# Autodesk Inventor assembly: 自動販賣機3.1
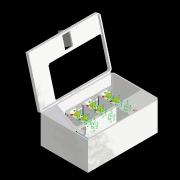
[picture p0: Inventor's stored thumbnail of the model, 180x180]
Saved by Autodesk Inventor 2020 (Build 240168000, 168)
## iProperties
Created: 2021-04-08
Part Number: 自動販賣機3.1
Document SubType Name: Assembly
Designer: 88690
Author: 88690
## Documents named in this file (33)
- C:\Users\88690\Desktop\自動販賣機\自動販賣機3.1.iam
- C:\Users\88690\Desktop\自動販賣機\上滑軌.ipt
- C:\Users\88690\Desktop\自動販賣機\上滑軌輪.ipt
- C:\Users\88690\Desktop\自動販賣機\下滑軌.ipt
- C:\Users\88690\Desktop\自動販賣機\下滑軌輪.ipt
- C:\Users\88690\Desktop\自動販賣機\本體.ipt
- C:\Users\88690\Desktop\自動販賣機\置物架.ipt
- C:\Users\88690\Desktop\自動販賣機\滾筒.ipt
- C:\Users\88690\Desktop\自動販賣機\蓋.ipt
- C:\Users\88690\Desktop\自動販賣機\鎖點支架.ipt
- C:\Users\88690\Desktop\自動販賣機\下支架右.ipt
- C:\Users\88690\Desktop\自動販賣機\上滑軌右.ipt
- C:\Users\88690\Desktop\自動販賣機\蝸桿支架.ipt
- C:\Users\88690\Desktop\自動販賣機\蝸桿滑塊.ipt
- C:\Users\88690\Desktop\自動販賣機\短蝸桿.ipt
- C:\Users\88690\Desktop\自動販賣機\長蝸桿.ipt
- C:\Users\88690\Desktop\自動販賣機\位移平台.ipt
- C:\Users\88690\Desktop\自動販賣機\取物窗.ipt
- C:\Users\88690\Desktop\自動販賣機\螺旋鉤子.ipt
- C:\Users\88690\Desktop\自動販賣機\螺旋鉤子底座.ipt
- C:\Users\88690\Desktop\自動販賣機\名牌1.ipt
- C:\Users\88690\Desktop\自動販賣機\名牌2.ipt
- C:\Users\88690\Desktop\自動販賣機\名牌3.ipt
- C:\Users\88690\Desktop\自動販賣機\名牌4.ipt
- C:\Users\88690\Desktop\自動販賣機\名牌5.ipt
- C:\Users\88690\Desktop\自動販賣機\名牌6.ipt
- C:\Users\88690\Desktop\自動販賣機\名牌7.ipt
- C:\Users\88690\Desktop\自動販賣機\名牌8.ipt
- C:\Users\88690\Desktop\自動販賣機\名牌9.ipt
- C:\Users\88690\Desktop\自動販賣機\模擬商品.ipt
- C:\Users\88690\Desktop\自動販賣機\模擬錢幣.ipt
- C:\Users\88690\Desktop\自動販賣機\路徑2.0.ipt
- C:\Users\88690\Desktop\自動販賣機\商品支架.ipt
## Components (117 placed, 32 different names)
1. 上滑軌:1 — 貼合:41, 貼合:42, 貼合:45, 相切:7, 貼合:183
2. 上滑軌輪:1 — 貼合:41, 貼合:42, 相切:1
3. 下滑軌:1 — 貼合:11, 貼合:12, 貼合:13, 貼合:15, 相切:1, 角度:40
4. 下滑軌輪:1 — 貼合:11, 貼合:12, 相切:7
5. 本體:1 — 齊平:1, 齊平:2, 齊平:3, 貼合:1, 貼合:2, 貼合:3, 貼合:4, 貼合:6, 貼合:7, 貼合:8, 貼合:9, 貼合:75, 貼合:76, 貼合:77, 貼合:78, 貼合:79, 貼合:80, 貼合:81, 貼合:82, 貼合:83, 貼合:84, 貼合:85, 貼合:86, 貼合:88, 貼合:89, 貼合:101, 齊平:23, 角度:1, 旋轉:1, 貼合:167, 角度:34, 貼合:169, 貼合:171, 貼合:172, 貼合:174, 齊平:50, 齊平:51, 貼合:177, 貼合:179, 齊平:53
6. 置物架:1 — 貼合:45, 貼合:50, 貼合:51, 齊平:12, 齊平:13, 貼合:111, 貼合:114, 貼合:131, 貼合:132, 貼合:139, 貼合:143, 貼合:144, 貼合:145, 貼合:146, 旋轉:2, 旋轉:3, 旋轉:10, 齊平:53, 齊平:54, 角度:40, 貼合:183, 角度:41, 貼合:187, 貼合:218, 貼合:219, 貼合:220, 貼合:221, 貼合:222, 貼合:223, 貼合:224
7. 滾筒:1 — 貼合:75, 貼合:76, 齊平:14, 齊平:15, 齊平:16, 齊平:17, 齊平:18, 齊平:19, 齊平:20, 齊平:21, 齊平:22, 角度:12, 旋轉:1, 旋轉:1, 貼合:178, 貼合:180
8. 蓋:1 — 貼合:101, 齊平:23, 角度:1, 角度:2, 貼合:108, 貼合:164, 角度:34, 角度:35
9. 鎖點支架:1 — 貼合:1, 貼合:2, 貼合:3, 齊平:4, 齊平:5, 齊平:6, 齊平:7, 貼合:5, 貼合:15, 貼合:22, 貼合:25
10. 鎖點支架:2 — 齊平:5, 齊平:7, 貼合:5, 貼合:13, 貼合:20, 貼合:23, 貼合:51, 貼合:72, 貼合:165, 貼合:166
11. 鎖點支架:3 — 齊平:4, 齊平:6, 貼合:4
12. 鎖點支架:4 — 齊平:8, 齊平:10, 貼合:9
13. 鎖點支架:5 — 貼合:6, 貼合:7, 貼合:8, 齊平:8, 齊平:9, 齊平:10, 齊平:11, 貼合:10, 貼合:30, 貼合:37, 貼合:40
14. 鎖點支架:6 — 齊平:9, 齊平:11, 貼合:10, 貼合:28, 貼合:35, 貼合:38
15. 下滑軌:2 — 貼合:20, 貼合:22, 相切:4
16. 下滑軌輪:2 — 相切:8
17. 下滑軌:3 — 貼合:23, 貼合:25, 相切:6
18. 下滑軌輪:3 — 相切:9
19. 下支架右:1 — 貼合:26, 貼合:27, 貼合:28, 貼合:30, 相切:2, 貼合:74, 角度:41
20. 下滑軌輪:4 — 貼合:26, 貼合:27, 相切:10
21. 下支架右:2 — 貼合:35, 貼合:37, 相切:3, 角度:42
22. 下滑軌輪:5 — 相切:11
23. 下支架右:3 — 貼合:38, 貼合:40, 相切:5, 角度:43
24. 下滑軌輪:6 — 相切:12
25. 上滑軌右:1 — 貼合:46, 貼合:50, 相切:10, 貼合:186, 貼合:187
26. 上滑軌輪:2 — 貼合:46, 相切:2, 貼合:74, 貼合:186
27. 上滑軌:2 — 相切:8, 貼合:184
28. 上滑軌輪:3 — 相切:4
29. 置物架:2 — 齊平:12, 貼合:72, 貼合:133, 貼合:134, 貼合:135, 貼合:140, 貼合:147, 貼合:150, 貼合:151, 貼合:152, 旋轉:4, 旋轉:5, 旋轉:9, 貼合:165, 齊平:54, 齊平:55, 貼合:184, 角度:42, 貼合:188, 貼合:225, 貼合:226, 貼合:227, 貼合:228, 貼合:229, 貼合:230
30. 上滑軌右:2 — 相切:11, 貼合:188
31. 上滑軌輪:4 — 相切:3
32. 上滑軌:3 — 相切:9, 貼合:185
33. 上滑軌輪:5 — 相切:6
34. 置物架:3 — 齊平:13, 貼合:136, 貼合:137, 貼合:138, 貼合:141, 貼合:148, 貼合:149, 貼合:153, 貼合:154, 旋轉:6, 旋轉:7, 旋轉:8, 貼合:166, 齊平:55, 貼合:185, 角度:43, 貼合:189, 貼合:231, 貼合:232, 貼合:233, 貼合:234, 貼合:235, 貼合:236
35. 上滑軌右:3 — 相切:12, 貼合:189
36. 上滑軌輪:6 — 相切:5
37. 滾筒:2 — 齊平:14, 貼合:77, 旋轉:1, 旋轉:2, 角度:13
38. 滾筒:3 — 齊平:15, 貼合:78, 旋轉:2, 角度:14, 旋轉:3
39. 滾筒:4 — 齊平:16, 貼合:79, 角度:15, 旋轉:3, 旋轉:4
40. 滾筒:5 — 齊平:17, 貼合:80, 角度:16, 旋轉:4, 旋轉:5
41. 滾筒:6 — 齊平:18, 貼合:81, 角度:18, 旋轉:5, 旋轉:6
42. 滾筒:7 — 齊平:19, 貼合:82, 角度:19, 旋轉:6, 旋轉:7
43. 滾筒:8 — 齊平:20, 貼合:83, 角度:22, 旋轉:7, 旋轉:8
44. 滾筒:9 — 齊平:21, 貼合:84, 角度:20, 旋轉:8, 旋轉:9
45. 滾筒:10 — 齊平:22, 貼合:85, 角度:21, 旋轉:9
46. 蝸桿支架:1 — 貼合:86, 貼合:88, 貼合:89, 貼合:90, 貼合:91, 貼合:92, 貼合:93
47. 蝸桿滑塊:1 — 貼合:90, 貼合:91, 貼合:94, 貼合:95, 貼合:97, 貼合:98, 貼合:99
48. 短蝸桿:1 — 貼合:94, 貼合:95, 旋轉/轉換:1
49. 長蝸桿:1 — 貼合:92, 貼合:93, 角度:23, 旋轉/轉換:1
50. 位移平台:1 — 貼合:97, 貼合:98, 貼合:99, 貼合:167, 貼合:182
51. 取物窗:1 — 角度:2, 貼合:108, 貼合:164, 角度:35
52. 螺旋鉤子:1 — 貼合:111, 貼合:112, 貼合:113, 角度:3, 貼合:155, 貼合:191, 貼合:199, 貼合:209
53. 螺旋鉤子底座:1 — 貼合:112, 貼合:113, 貼合:114, 貼合:155, 旋轉:2
54. 螺旋鉤子:2 — 貼合:131, 齊平:44, 貼合:190, 貼合:198, 貼合:208
55. 螺旋鉤子底座:2 — 齊平:25, 貼合:139, 齊平:44, 旋轉:3
56. 螺旋鉤子:3 — 貼合:132, 齊平:47, 貼合:197, 貼合:200, 貼合:210
57. 螺旋鉤子底座:3 — 齊平:25, 齊平:47, 旋轉:10
58. 螺旋鉤子:4 — 貼合:133, 貼合:157, 貼合:192, 貼合:201, 貼合:211, 齊平:96
59. 螺旋鉤子底座:4 — 齊平:26, 齊平:27, 貼合:140, 貼合:157, 旋轉:4
60. 螺旋鉤子:5 — 貼合:134, 貼合:158, 貼合:168, 貼合:170, 角度:37, 齊平:49, 貼合:202, 貼合:207, 貼合:212, 貼合:217, 齊平:96
61. 螺旋鉤子底座:5 — 齊平:26, 貼合:158, 旋轉:5
62. 螺旋鉤子:6 — 貼合:135, 齊平:46, 貼合:193, 貼合:203, 貼合:213
63. 螺旋鉤子底座:6 — 齊平:27, 齊平:46, 旋轉:9
64. 螺旋鉤子:7 — 貼合:136, 貼合:160, 貼合:194, 貼合:204, 貼合:214
65. 螺旋鉤子底座:7 — 齊平:28, 齊平:29, 貼合:141, 貼合:160, 旋轉:6
66. 螺旋鉤子:8 — 貼合:137, 貼合:161, 貼合:195, 貼合:205, 貼合:215
67. 螺旋鉤子底座:8 — 齊平:28, 貼合:161, 旋轉:7
68. 螺旋鉤子:9 — 貼合:138, 齊平:45, 貼合:196, 貼合:206, 貼合:216
69. 螺旋鉤子底座:9 — 齊平:29, 齊平:45, 旋轉:8
70. 名牌1:1 — 貼合:143, 貼合:144, 角度:24, 齊平:30, 角度:25, 角度:29
71. 名牌2:1 — 貼合:145, 齊平:30, 齊平:31, 角度:25, 角度:26
72. 名牌3:1 — 貼合:146, 齊平:31, 角度:26
73. 名牌4:1 — 齊平:32, 齊平:33, 貼合:147, 貼合:150, 角度:27, 角度:28, 角度:29
74. 名牌5:1 — 齊平:32, 貼合:151, 角度:27
75. 名牌6:1 — 齊平:33, 貼合:152, 角度:32
76. 名牌7:1 — 齊平:34, 貼合:148, 貼合:149, 角度:28
77. 名牌8:1 — 齊平:34, 齊平:35, 貼合:153, 角度:30
78. 名牌9:1 — 齊平:35, 貼合:154, 角度:33
79. 模擬商品:1 — 貼合:168, 角度:36, 貼合:170, 角度:38, 貼合:176, 貼合:177, 貼合:178, 貼合:181, 貼合:182, 齊平:63
80. 模擬錢幣:1 — 貼合:169, 貼合:171, 貼合:172
81. 路徑2.0:1 — 貼合:174, 貼合:176, 角度:39, 齊平:50, 齊平:51
82. 路徑2.0:2 — 貼合:179, 貼合:180, 齊平:52, 貼合:181
83. 模擬商品:2 — 貼合:190, 齊平:56, 齊平:57, 齊平:58, 齊平:59, 齊平:60, 齊平:61, 齊平:62, 齊平:63
84. 模擬商品:3 — 貼合:191, 齊平:56
85. 模擬商品:4 — 貼合:192, 齊平:58
86. 模擬商品:5 — 貼合:193, 齊平:59
87. 模擬商品:6 — 貼合:194, 齊平:62
88. 模擬商品:7 — 貼合:197, 齊平:57
89. 模擬商品:8 — 貼合:195, 齊平:61
90. 模擬商品:9 — 貼合:196, 齊平:60
91. 模擬商品:10 — 齊平:83, 貼合:202, 貼合:207
92. 模擬商品:11 — 齊平:80, 齊平:81, 齊平:82, 齊平:83, 齊平:84, 齊平:85, 齊平:86, 齊平:87, 貼合:198
93. 模擬商品:12 — 齊平:80, 貼合:199
94. 模擬商品:13 — 齊平:82, 貼合:201
95. 模擬商品:14 — 齊平:84, 貼合:203
96. 模擬商品:15 — 齊平:85, 貼合:204
97. 模擬商品:16 — 齊平:81, 貼合:200
98. 模擬商品:17 — 齊平:86, 貼合:205
99. 模擬商品:18 — 齊平:87, 貼合:206
100. 模擬商品:19 — 齊平:91, 貼合:212, 貼合:217
101. 模擬商品:20 — 齊平:88, 齊平:90, 齊平:91, 齊平:92, 齊平:93, 齊平:94, 齊平:95, 貼合:208
102. 模擬商品:21 — 齊平:88, 齊平:89, 貼合:209
103. 模擬商品:22 — 齊平:90, 貼合:211
104. 模擬商品:23 — 齊平:92, 貼合:213
105. 模擬商品:24 — 齊平:93, 貼合:214
106. 模擬商品:25 — 齊平:89, 貼合:210
107. 模擬商品:26 — 齊平:94, 貼合:215
108. 模擬商品:27 — 齊平:95, 貼合:216
109. 商品支架:1 — 貼合:218, 貼合:219, 貼合:220, 齊平:103
110. 商品支架:2 — 齊平:97, 貼合:221, 貼合:222, 齊平:103, 齊平:104
111. 商品支架:3 — 齊平:97, 齊平:98, 貼合:225, 貼合:226
112. 商品支架:4 — 齊平:98, 齊平:99, 貼合:235, 貼合:236
113. 商品支架:5 — 齊平:99, 齊平:100, 貼合:227, 貼合:228
114. 商品支架:6 — 齊平:100, 齊平:101, 貼合:229, 貼合:230
115. 商品支架:7 — 齊平:101, 齊平:102, 貼合:231, 貼合:232
116. 商品支架:8 — 貼合:223, 貼合:224, 齊平:104
117. 商品支架:9 — 齊平:102, 貼合:233, 貼合:234
## Relationships (357: Mate 198, Flush 94, Angle 33, Tangent 12, RevoluteJoint 10, RelateRotation 9, RelateRotateTranslate 1)
- 齊平:1 [Flush]: 本體:1
- 齊平:2 [Flush]: 本體:1
- 齊平:3 [Flush]: 本體:1
- 貼合:1 [Mate] (180 mm): 本體:1 ↔ 鎖點支架:1
- 貼合:2 [Mate]: 本體:1 ↔ 鎖點支架:1
- 貼合:3 [Mate]: 本體:1 ↔ 鎖點支架:1
- 齊平:4 [Flush]: 鎖點支架:1 ↔ 鎖點支架:3
- 齊平:5 [Flush]: 鎖點支架:1 ↔ 鎖點支架:2
- 齊平:6 [Flush]: 鎖點支架:1 ↔ 鎖點支架:3
- 齊平:7 [Flush]: 鎖點支架:1 ↔ 鎖點支架:2
- 貼合:4 [Mate]: 本體:1 ↔ 鎖點支架:3
- 貼合:5 [Mate] (55 mm): 鎖點支架:1 ↔ 鎖點支架:2
- 貼合:6 [Mate]: 本體:1 ↔ 鎖點支架:5
- 貼合:7 [Mate]: 本體:1 ↔ 鎖點支架:5
- 貼合:8 [Mate] (180 mm): 本體:1 ↔ 鎖點支架:5
- 齊平:8 [Flush]: 鎖點支架:4 ↔ 鎖點支架:5
- 齊平:9 [Flush]: 鎖點支架:5 ↔ 鎖點支架:6
- 齊平:10 [Flush]: 鎖點支架:4 ↔ 鎖點支架:5
- 齊平:11 [Flush]: 鎖點支架:5 ↔ 鎖點支架:6
- 貼合:9 [Mate]: 本體:1 ↔ 鎖點支架:4
- 貼合:10 [Mate] (55 mm): 鎖點支架:5 ↔ 鎖點支架:6
- 貼合:11 [Mate]: 下滑軌:1 ↔ 下滑軌輪:1
- 貼合:12 [Mate]: 下滑軌:1 ↔ 下滑軌輪:1
- 貼合:13 [Mate]: 下滑軌:1 ↔ 鎖點支架:2
- 貼合:15 [Mate]: 下滑軌:1 ↔ 鎖點支架:1
- [Mate]: 下滑軌:2 ↔ 下滑軌輪:2
- [Mate]: 下滑軌:2 ↔ 下滑軌輪:2
- [Mate]: 下滑軌:3 ↔ 下滑軌輪:3
- [Mate]: 下滑軌:3 ↔ 下滑軌輪:3
- 貼合:20 [Mate]: 鎖點支架:2 ↔ 下滑軌:2
- 貼合:22 [Mate]: 鎖點支架:1 ↔ 下滑軌:2
- 貼合:23 [Mate]: 鎖點支架:2 ↔ 下滑軌:3
- 貼合:25 [Mate]: 鎖點支架:1 ↔ 下滑軌:3
- 貼合:26 [Mate]: 下支架右:1 ↔ 下滑軌輪:4
- 貼合:27 [Mate]: 下支架右:1 ↔ 下滑軌輪:4
- 貼合:28 [Mate]: 鎖點支架:6 ↔ 下支架右:1
- 貼合:30 [Mate]: 鎖點支架:5 ↔ 下支架右:1
- [Mate]: 下支架右:2 ↔ 下滑軌輪:5
- [Mate]: 下支架右:2 ↔ 下滑軌輪:5
- [Mate]: 下支架右:3 ↔ 下滑軌輪:6
- [Mate]: 下支架右:3 ↔ 下滑軌輪:6
- 貼合:35 [Mate]: 鎖點支架:6 ↔ 下支架右:2
- 貼合:37 [Mate]: 鎖點支架:5 ↔ 下支架右:2
- 貼合:38 [Mate]: 鎖點支架:6 ↔ 下支架右:3
- 貼合:40 [Mate]: 鎖點支架:5 ↔ 下支架右:3
- 貼合:41 [Mate]: 上滑軌:1 ↔ 上滑軌輪:1
- 貼合:42 [Mate]: 上滑軌:1 ↔ 上滑軌輪:1
- 貼合:45 [Mate]: 上滑軌:1 ↔ 置物架:1
- 貼合:46 [Mate]: 上滑軌右:1 ↔ 上滑軌輪:2
- 貼合:50 [Mate]: 置物架:1 ↔ 上滑軌右:1
- 相切:1 [Tangent]: 上滑軌輪:1 ↔ 下滑軌:1
- 相切:2 [Tangent]: 下支架右:1 ↔ 上滑軌輪:2
- 貼合:51 [Mate]: 置物架:1 ↔ 鎖點支架:2
- [Mate]: 上滑軌:2 ↔ 上滑軌輪:3
- [Mate]: 上滑軌:2 ↔ 上滑軌輪:3
- [Mate]: 上滑軌:2 ↔ 置物架:2
- [Mate]: 上滑軌右:2 ↔ 上滑軌輪:4
- [Mate]: 上滑軌右:2 ↔ 上滑軌輪:4
- [Mate]: 置物架:2 ↔ 上滑軌右:2
- [Mate]: 上滑軌:3 ↔ 上滑軌輪:5
- [Mate]: 上滑軌:3 ↔ 上滑軌輪:5
- [Mate]: 上滑軌:3 ↔ 置物架:3
- [Mate]: 上滑軌右:3 ↔ 上滑軌輪:6
- [Mate]: 上滑軌右:3 ↔ 上滑軌輪:6
- [Mate]: 置物架:3 ↔ 上滑軌右:3
- 齊平:12 [Flush]: 置物架:1 ↔ 置物架:2
- 齊平:13 [Flush]: 置物架:1 ↔ 置物架:3
- 相切:3 [Tangent]: 下支架右:2 ↔ 上滑軌輪:4
- 相切:4 [Tangent]: 下滑軌:2 ↔ 上滑軌輪:3
- 相切:5 [Tangent]: 下支架右:3 ↔ 上滑軌輪:6
- 相切:6 [Tangent]: 下滑軌:3 ↔ 上滑軌輪:5
- 貼合:72 [Mate] (150 mm): 鎖點支架:2 ↔ 置物架:2
- 貼合:74 [Mate]: 下支架右:1 ↔ 上滑軌輪:2
- 貼合:75 [Mate]: 本體:1 ↔ 滾筒:1
- 貼合:76 [Mate]: 本體:1 ↔ 滾筒:1
- 齊平:14 [Flush]: 滾筒:1 ↔ 滾筒:2
- 齊平:15 [Flush]: 滾筒:1 ↔ 滾筒:3
- 齊平:16 [Flush]: 滾筒:1 ↔ 滾筒:4
- 齊平:17 [Flush]: 滾筒:1 ↔ 滾筒:5
- 齊平:18 [Flush]: 滾筒:1 ↔ 滾筒:6
- 齊平:19 [Flush]: 滾筒:1 ↔ 滾筒:7
- 齊平:20 [Flush]: 滾筒:1 ↔ 滾筒:8
- 齊平:21 [Flush]: 滾筒:1 ↔ 滾筒:9
- 齊平:22 [Flush]: 滾筒:1 ↔ 滾筒:10
- 貼合:77 [Mate]: 本體:1 ↔ 滾筒:2
- 貼合:78 [Mate]: 本體:1 ↔ 滾筒:3
- 貼合:79 [Mate]: 本體:1 ↔ 滾筒:4
- 貼合:80 [Mate]: 本體:1 ↔ 滾筒:5
- 貼合:81 [Mate]: 本體:1 ↔ 滾筒:6
- 貼合:82 [Mate]: 本體:1 ↔ 滾筒:7
- 貼合:83 [Mate]: 本體:1 ↔ 滾筒:8
- 貼合:84 [Mate]: 本體:1 ↔ 滾筒:9
- 貼合:85 [Mate]: 本體:1 ↔ 滾筒:10
- 貼合:86 [Mate]: 本體:1 ↔ 蝸桿支架:1
- 貼合:88 [Mate]: 本體:1 ↔ 蝸桿支架:1
- 貼合:89 [Mate]: 本體:1 ↔ 蝸桿支架:1
- 貼合:90 [Mate]: 蝸桿支架:1 ↔ 蝸桿滑塊:1
- 貼合:91 [Mate]: 蝸桿支架:1 ↔ 蝸桿滑塊:1
- 貼合:92 [Mate]: 蝸桿支架:1 ↔ 長蝸桿:1
- 貼合:93 [Mate]: 蝸桿支架:1 ↔ 長蝸桿:1
- 貼合:94 [Mate]: 蝸桿滑塊:1 ↔ 短蝸桿:1
- 貼合:95 [Mate]: 蝸桿滑塊:1 ↔ 短蝸桿:1
- 貼合:97 [Mate]: 蝸桿滑塊:1 ↔ 位移平台:1
- 貼合:98 [Mate]: 蝸桿滑塊:1 ↔ 位移平台:1
- 貼合:99 [Mate]: 蝸桿滑塊:1 ↔ 位移平台:1
- 貼合:101 [Mate]: 本體:1 ↔ 蓋:1
- 齊平:23 [Flush]: 本體:1 ↔ 蓋:1
- 角度:1 [Angle] (45 deg): 本體:1 ↔ 蓋:1
- 角度:2 [Angle] (180 deg): 蓋:1 ↔ 取物窗:1
- 貼合:108 [Mate]: 蓋:1 ↔ 取物窗:1
- 貼合:111 [Mate]: 置物架:1 ↔ 螺旋鉤子:1
- 貼合:112 [Mate]: 螺旋鉤子:1 ↔ 螺旋鉤子底座:1
- 貼合:113 [Mate]: 螺旋鉤子:1 ↔ 螺旋鉤子底座:1
- 角度:3 [Angle] (0 deg): 螺旋鉤子:1
- 貼合:114 [Mate]: 置物架:1 ↔ 螺旋鉤子底座:1
- [Mate]: 螺旋鉤子:2 ↔ 螺旋鉤子底座:2
- [Mate]: 螺旋鉤子:2 ↔ 螺旋鉤子底座:2
- [Mate]: 螺旋鉤子:3 ↔ 螺旋鉤子底座:3
- [Mate]: 螺旋鉤子:3 ↔ 螺旋鉤子底座:3
- [Mate]: 螺旋鉤子:4 ↔ 螺旋鉤子底座:4
- [Mate]: 螺旋鉤子:4 ↔ 螺旋鉤子底座:4
- [Mate]: 螺旋鉤子:5 ↔ 螺旋鉤子底座:5
- [Mate]: 螺旋鉤子:5 ↔ 螺旋鉤子底座:5
- [Mate]: 螺旋鉤子:6 ↔ 螺旋鉤子底座:6
- [Mate]: 螺旋鉤子:6 ↔ 螺旋鉤子底座:6
- [Mate]: 螺旋鉤子:7 ↔ 螺旋鉤子底座:7
- [Mate]: 螺旋鉤子:7 ↔ 螺旋鉤子底座:7
- [Mate]: 螺旋鉤子:8 ↔ 螺旋鉤子底座:8
- [Mate]: 螺旋鉤子:8 ↔ 螺旋鉤子底座:8
- [Mate]: 螺旋鉤子:9 ↔ 螺旋鉤子底座:9
- [Mate]: 螺旋鉤子:9 ↔ 螺旋鉤子底座:9
- 齊平:25 [Flush]: 螺旋鉤子底座:2 ↔ 螺旋鉤子底座:3
- 貼合:131 [Mate]: 置物架:1 ↔ 螺旋鉤子:2
- 貼合:132 [Mate]: 置物架:1 ↔ 螺旋鉤子:3
- 貼合:133 [Mate]: 置物架:2 ↔ 螺旋鉤子:4
- 貼合:134 [Mate]: 置物架:2 ↔ 螺旋鉤子:5
- 貼合:135 [Mate]: 置物架:2 ↔ 螺旋鉤子:6
- 貼合:136 [Mate]: 置物架:3 ↔ 螺旋鉤子:7
- 貼合:137 [Mate]: 置物架:3 ↔ 螺旋鉤子:8
- 貼合:138 [Mate]: 置物架:3 ↔ 螺旋鉤子:9
- 貼合:139 [Mate]: 置物架:1 ↔ 螺旋鉤子底座:2
- 齊平:26 [Flush]: 螺旋鉤子底座:4 ↔ 螺旋鉤子底座:5
- 齊平:27 [Flush]: 螺旋鉤子底座:4 ↔ 螺旋鉤子底座:6
- 齊平:28 [Flush]: 螺旋鉤子底座:7 ↔ 螺旋鉤子底座:8
- 齊平:29 [Flush]: 螺旋鉤子底座:7 ↔ 螺旋鉤子底座:9
- 貼合:140 [Mate]: 置物架:2 ↔ 螺旋鉤子底座:4
- 貼合:141 [Mate]: 置物架:3 ↔ 螺旋鉤子底座:7
- 角度:12 [Angle] (4455 deg): 滾筒:1
- 旋轉:1 [RelateRotation] (1 ul): 滾筒:1 ↔ 滾筒:2
- 旋轉:2 [RelateRotation] (1 ul): 滾筒:2 ↔ 滾筒:3
- 角度:13 [Angle] (135 deg): 滾筒:2
- 角度:14 [Angle] (135 deg): 滾筒:3
- 角度:15 [Angle] (135 deg): 滾筒:4
- 角度:16 [Angle] (135 deg): 滾筒:5
- 角度:18 [Angle] (135 deg): 滾筒:6
- 角度:19 [Angle] (135 deg): 滾筒:7
- 角度:20 [Angle] (135 deg): 滾筒:9
- 角度:21 [Angle] (135 deg): 滾筒:10
- 角度:22 [Angle] (135 deg): 滾筒:8
- 旋轉:3 [RelateRotation] (1 ul): 滾筒:3 ↔ 滾筒:4
- 旋轉:4 [RelateRotation] (1 ul): 滾筒:4 ↔ 滾筒:5
- 旋轉:5 [RelateRotation] (1 ul): 滾筒:5 ↔ 滾筒:6
- 旋轉:6 [RelateRotation] (1 ul): 滾筒:6 ↔ 滾筒:7
- 旋轉:7 [RelateRotation] (1 ul): 滾筒:7 ↔ 滾筒:8
- 旋轉:8 [RelateRotation] (1 ul): 滾筒:8 ↔ 滾筒:9
- 旋轉:9 [RelateRotation] (1 ul): 滾筒:9 ↔ 滾筒:10
- 旋轉:1 [RevoluteJoint]: 本體:1 ↔ 滾筒:1
- 角度:23 [Angle] (0 deg): 長蝸桿:1
- 旋轉/轉換:1 [RelateRotateTranslate] (103.673 mm): 短蝸桿:1 ↔ 長蝸桿:1
- 貼合:143 [Mate]: 置物架:1 ↔ 名牌1:1
- 貼合:144 [Mate]: 置物架:1 ↔ 名牌1:1
- 角度:24 [Angle] (0 deg): 名牌1:1
- 貼合:145 [Mate]: 置物架:1 ↔ 名牌2:1
- 貼合:146 [Mate]: 置物架:1 ↔ 名牌3:1
- 齊平:30 [Flush]: 名牌1:1 ↔ 名牌2:1
- 齊平:31 [Flush]: 名牌2:1 ↔ 名牌3:1
- 齊平:32 [Flush]: 名牌4:1 ↔ 名牌5:1
- 齊平:33 [Flush]: 名牌4:1 ↔ 名牌6:1
- 齊平:34 [Flush]: 名牌7:1 ↔ 名牌8:1
- 齊平:35 [Flush]: 名牌8:1 ↔ 名牌9:1
- 貼合:147 [Mate]: 置物架:2 ↔ 名牌4:1
- 貼合:148 [Mate]: 置物架:3 ↔ 名牌7:1
- 貼合:149 [Mate]: 置物架:3 ↔ 名牌7:1
- 貼合:150 [Mate]: 置物架:2 ↔ 名牌4:1
- 貼合:151 [Mate]: 置物架:2 ↔ 名牌5:1
- 貼合:152 [Mate]: 置物架:2 ↔ 名牌6:1
- 貼合:153 [Mate]: 置物架:3 ↔ 名牌8:1
- 角度:25 [Angle] (0 deg): 名牌1:1 ↔ 名牌2:1
- 角度:26 [Angle] (0 deg): 名牌2:1 ↔ 名牌3:1
- 角度:27 [Angle] (0 deg): 名牌4:1 ↔ 名牌5:1
- 角度:28 [Angle] (0 deg): 名牌4:1 ↔ 名牌7:1
- 角度:29 [Angle] (0 deg): 名牌1:1 ↔ 名牌4:1
- 貼合:154 [Mate]: 置物架:3 ↔ 名牌9:1
- 角度:30 [Angle] (0 deg): 名牌8:1
- 角度:32 [Angle] (0 deg): 名牌6:1
- 角度:33 [Angle] (0 deg): 名牌9:1
- 貼合:155 [Mate]: 螺旋鉤子:1 ↔ 螺旋鉤子底座:1
- 旋轉:2 [RevoluteJoint]: 置物架:1 ↔ 螺旋鉤子底座:1
- 齊平:44 [Flush]: 螺旋鉤子:2 ↔ 螺旋鉤子底座:2
- 旋轉:3 [RevoluteJoint]: 置物架:1 ↔ 螺旋鉤子底座:2
- 貼合:157 [Mate]: 螺旋鉤子:4 ↔ 螺旋鉤子底座:4
- 旋轉:4 [RevoluteJoint]: 置物架:2 ↔ 螺旋鉤子底座:4
- 貼合:158 [Mate]: 螺旋鉤子:5 ↔ 螺旋鉤子底座:5
- 旋轉:5 [RevoluteJoint]: 置物架:2 ↔ 螺旋鉤子底座:5
- 貼合:160 [Mate]: 螺旋鉤子:7 ↔ 螺旋鉤子底座:7
- 旋轉:6 [RevoluteJoint]: 置物架:3 ↔ 螺旋鉤子底座:7
- 貼合:161 [Mate]: 螺旋鉤子:8 ↔ 螺旋鉤子底座:8
- 旋轉:7 [RevoluteJoint]: 置物架:3 ↔ 螺旋鉤子底座:8
- 齊平:45 [Flush]: 螺旋鉤子:9 ↔ 螺旋鉤子底座:9
- 旋轉:8 [RevoluteJoint]: 置物架:3 ↔ 螺旋鉤子底座:9
- 齊平:46 [Flush]: 螺旋鉤子:6 ↔ 螺旋鉤子底座:6
- 旋轉:9 [RevoluteJoint]: 置物架:2 ↔ 螺旋鉤子底座:6
- 齊平:47 [Flush]: 螺旋鉤子:3 ↔ 螺旋鉤子底座:3
- 旋轉:10 [RevoluteJoint]: 置物架:1 ↔ 螺旋鉤子底座:3
- 貼合:164 [Mate]: 蓋:1 ↔ 取物窗:1
- 貼合:165 [Mate]: 鎖點支架:2 ↔ 置物架:2
- 貼合:166 [Mate]: 鎖點支架:2 ↔ 置物架:3
- 貼合:167 [Mate]: 本體:1 ↔ 位移平台:1
- 角度:34 [Angle] (75 deg): 本體:1 ↔ 蓋:1
- 角度:35 [Angle] (135 deg): 蓋:1 ↔ 取物窗:1
- 貼合:168 [Mate]: 螺旋鉤子:5 ↔ 模擬商品:1
- 貼合:169 [Mate] (0.5 mm): 本體:1 ↔ 模擬錢幣:1
- 角度:36 [Angle] (-15 deg): 模擬商品:1
- 貼合:170 [Mate]: 螺旋鉤子:5 ↔ 模擬商品:1
- 貼合:171 [Mate]: 本體:1 ↔ 模擬錢幣:1
- 貼合:172 [Mate] (150 mm): 本體:1 ↔ 模擬錢幣:1
- 角度:37 [Angle] (-360 deg): 螺旋鉤子:5
- 角度:38 [Angle] (0 deg): 模擬商品:1
- 齊平:49 [Flush]: 螺旋鉤子:5
- 貼合:174 [Mate]: 本體:1 ↔ 路徑2.0:1
- 貼合:176 [Mate]: 模擬商品:1 ↔ 路徑2.0:1
- 角度:39 [Angle] (0 deg): 路徑2.0:1
- 齊平:50 [Flush]: 本體:1 ↔ 路徑2.0:1
- 齊平:51 [Flush]: 本體:1 ↔ 路徑2.0:1
- 貼合:177 [Mate]: 本體:1 ↔ 模擬商品:1
- 貼合:178 [Mate]: 滾筒:1 ↔ 模擬商品:1
- 貼合:179 [Mate]: 本體:1 ↔ 路徑2.0:2
- 貼合:180 [Mate]: 滾筒:1 ↔ 路徑2.0:2
- 齊平:52 [Flush]: 路徑2.0:2
- 貼合:181 [Mate]: 模擬商品:1 ↔ 路徑2.0:2
- 貼合:182 [Mate]: 位移平台:1 ↔ 模擬商品:1
- 齊平:53 [Flush] (-390 mm): 本體:1 ↔ 置物架:1
- 齊平:54 [Flush] (400 mm): 置物架:1 ↔ 置物架:2
- 齊平:55 [Flush] (400 mm): 置物架:2 ↔ 置物架:3
- 角度:40 [Angle] (0 deg): 下滑軌:1 ↔ 置物架:1
- 相切:7 [Tangent]: 上滑軌:1 ↔ 下滑軌輪:1
- 貼合:183 [Mate]: 上滑軌:1 ↔ 置物架:1
- 相切:8 [Tangent]: 下滑軌輪:2 ↔ 上滑軌:2
- 貼合:184 [Mate]: 上滑軌:2 ↔ 置物架:2
- 相切:9 [Tangent]: 下滑軌輪:3 ↔ 上滑軌:3
- 貼合:185 [Mate]: 上滑軌:3 ↔ 置物架:3
- 角度:41 [Angle] (0 deg): 置物架:1 ↔ 下支架右:1
- 相切:10 [Tangent]: 下滑軌輪:4 ↔ 上滑軌右:1
- 貼合:186 [Mate]: 上滑軌右:1 ↔ 上滑軌輪:2
- 貼合:187 [Mate]: 置物架:1 ↔ 上滑軌右:1
- 角度:42 [Angle] (0 deg): 下支架右:2 ↔ 置物架:2
- 角度:43 [Angle] (0 deg): 下支架右:3 ↔ 置物架:3
- 相切:11 [Tangent]: 下滑軌輪:5 ↔ 上滑軌右:2
- 貼合:188 [Mate]: 置物架:2 ↔ 上滑軌右:2
- 相切:12 [Tangent]: 下滑軌輪:6 ↔ 上滑軌右:3
- 貼合:189 [Mate]: 置物架:3 ↔ 上滑軌右:3
- 貼合:190 [Mate]: 螺旋鉤子:2 ↔ 模擬商品:2
- 貼合:191 [Mate]: 螺旋鉤子:1 ↔ 模擬商品:3
- 貼合:192 [Mate]: 螺旋鉤子:4 ↔ 模擬商品:4
- 貼合:193 [Mate]: 螺旋鉤子:6 ↔ 模擬商品:5
- 貼合:194 [Mate]: 螺旋鉤子:7 ↔ 模擬商品:6
- 貼合:195 [Mate]: 螺旋鉤子:8 ↔ 模擬商品:8
- 貼合:196 [Mate]: 螺旋鉤子:9 ↔ 模擬商品:9
- 貼合:197 [Mate]: 螺旋鉤子:3 ↔ 模擬商品:7
- 齊平:56 [Flush]: 模擬商品:2 ↔ 模擬商品:3
- 齊平:57 [Flush]: 模擬商品:2 ↔ 模擬商品:7
- 齊平:58 [Flush]: 模擬商品:2 ↔ 模擬商品:4
- 齊平:59 [Flush]: 模擬商品:2 ↔ 模擬商品:5
- 齊平:60 [Flush]: 模擬商品:2 ↔ 模擬商品:9
- 齊平:61 [Flush]: 模擬商品:2 ↔ 模擬商品:8
- 齊平:62 [Flush]: 模擬商品:2 ↔ 模擬商品:6
- 齊平:63 [Flush]: 模擬商品:1 ↔ 模擬商品:2
- [Flush]: 模擬商品:11 ↔ 模擬商品:12
- [Flush]: 模擬商品:11 ↔ 模擬商品:16
- [Flush]: 模擬商品:11 ↔ 模擬商品:13
- [Flush]: 模擬商品:11 ↔ 模擬商品:14
- [Flush]: 模擬商品:11 ↔ 模擬商品:18
- [Flush]: 模擬商品:11 ↔ 模擬商品:17
- [Flush]: 模擬商品:11 ↔ 模擬商品:15
- [Flush]: 模擬商品:10 ↔ 模擬商品:11
- [Flush]: 模擬商品:20 ↔ 模擬商品:21
- [Flush]: 模擬商品:20 ↔ 模擬商品:25
- [Flush]: 模擬商品:20 ↔ 模擬商品:22
- [Flush]: 模擬商品:20 ↔ 模擬商品:23
- [Flush]: 模擬商品:20 ↔ 模擬商品:27
- [Flush]: 模擬商品:20 ↔ 模擬商品:26
- [Flush]: 模擬商品:20 ↔ 模擬商品:24
- [Flush]: 模擬商品:19 ↔ 模擬商品:20
- 齊平:80 [Flush]: 模擬商品:11 ↔ 模擬商品:12
- 齊平:81 [Flush]: 模擬商品:11 ↔ 模擬商品:16
- 齊平:82 [Flush]: 模擬商品:11 ↔ 模擬商品:13
- 齊平:83 [Flush]: 模擬商品:10 ↔ 模擬商品:11
- 齊平:84 [Flush]: 模擬商品:11 ↔ 模擬商品:14
- 齊平:85 [Flush]: 模擬商品:11 ↔ 模擬商品:15
- 齊平:86 [Flush]: 模擬商品:11 ↔ 模擬商品:17
- 齊平:87 [Flush]: 模擬商品:11 ↔ 模擬商品:18
- 齊平:88 [Flush]: 模擬商品:20 ↔ 模擬商品:21
- 齊平:89 [Flush]: 模擬商品:21 ↔ 模擬商品:25
- 齊平:90 [Flush]: 模擬商品:20 ↔ 模擬商品:22
- 齊平:91 [Flush]: 模擬商品:19 ↔ 模擬商品:20
- 齊平:92 [Flush]: 模擬商品:20 ↔ 模擬商品:23
- 齊平:93 [Flush]: 模擬商品:20 ↔ 模擬商品:24
- 齊平:94 [Flush]: 模擬商品:20 ↔ 模擬商品:26
- 齊平:95 [Flush]: 模擬商品:20 ↔ 模擬商品:27
- 貼合:198 [Mate]: 螺旋鉤子:2 ↔ 模擬商品:11
- 貼合:199 [Mate]: 螺旋鉤子:1 ↔ 模擬商品:12
- 貼合:200 [Mate]: 螺旋鉤子:3 ↔ 模擬商品:16
- 貼合:201 [Mate]: 螺旋鉤子:4 ↔ 模擬商品:13
- 貼合:202 [Mate]: 螺旋鉤子:5 ↔ 模擬商品:10
- 貼合:203 [Mate]: 螺旋鉤子:6 ↔ 模擬商品:14
- 貼合:204 [Mate]: 螺旋鉤子:7 ↔ 模擬商品:15
- 貼合:205 [Mate]: 螺旋鉤子:8 ↔ 模擬商品:17
- 貼合:206 [Mate]: 螺旋鉤子:9 ↔ 模擬商品:18
- 貼合:207 [Mate]: 螺旋鉤子:5 ↔ 模擬商品:10
- 貼合:208 [Mate]: 螺旋鉤子:2 ↔ 模擬商品:20
- 貼合:209 [Mate]: 螺旋鉤子:1 ↔ 模擬商品:21
- 貼合:210 [Mate]: 螺旋鉤子:3 ↔ 模擬商品:25
- 貼合:211 [Mate]: 螺旋鉤子:4 ↔ 模擬商品:22
- 貼合:212 [Mate]: 螺旋鉤子:5 ↔ 模擬商品:19
- 貼合:213 [Mate]: 螺旋鉤子:6 ↔ 模擬商品:23
- 貼合:214 [Mate]: 螺旋鉤子:7 ↔ 模擬商品:24
- 貼合:215 [Mate]: 螺旋鉤子:8 ↔ 模擬商品:26
- 貼合:216 [Mate]: 螺旋鉤子:9 ↔ 模擬商品:27
- 貼合:217 [Mate]: 螺旋鉤子:5 ↔ 模擬商品:19
- 齊平:96 [Flush]: 螺旋鉤子:4 ↔ 螺旋鉤子:5
- 貼合:218 [Mate]: 置物架:1 ↔ 商品支架:1
- 貼合:219 [Mate]: 置物架:1 ↔ 商品支架:1
- 貼合:220 [Mate]: 置物架:1 ↔ 商品支架:1
- 齊平:97 [Flush]: 商品支架:2 ↔ 商品支架:3
- 齊平:98 [Flush]: 商品支架:3 ↔ 商品支架:4
- 齊平:99 [Flush]: 商品支架:4 ↔ 商品支架:5
- 齊平:100 [Flush]: 商品支架:5 ↔ 商品支架:6
- 齊平:101 [Flush]: 商品支架:6 ↔ 商品支架:7
- 齊平:102 [Flush]: 商品支架:7 ↔ 商品支架:9
- 貼合:221 [Mate]: 置物架:1 ↔ 商品支架:2
- 貼合:222 [Mate]: 置物架:1 ↔ 商品支架:2
- 齊平:103 [Flush]: 商品支架:1 ↔ 商品支架:2
- 貼合:223 [Mate]: 置物架:1 ↔ 商品支架:8
- 貼合:224 [Mate]: 置物架:1 ↔ 商品支架:8
- 貼合:225 [Mate]: 置物架:2 ↔ 商品支架:3
- 貼合:226 [Mate]: 置物架:2 ↔ 商品支架:3
- 貼合:227 [Mate]: 置物架:2 ↔ 商品支架:5
- 貼合:228 [Mate]: 置物架:2 ↔ 商品支架:5
- 貼合:229 [Mate]: 置物架:2 ↔ 商品支架:6
- 貼合:230 [Mate]: 置物架:2 ↔ 商品支架:6
- 貼合:231 [Mate]: 置物架:3 ↔ 商品支架:7
- 貼合:232 [Mate]: 置物架:3 ↔ 商品支架:7
- 貼合:233 [Mate]: 置物架:3 ↔ 商品支架:9
- 貼合:234 [Mate]: 置物架:3 ↔ 商品支架:9
- 貼合:235 [Mate]: 置物架:3 ↔ 商品支架:4
- 貼合:236 [Mate]: 置物架:3 ↔ 商品支架:4
- 齊平:104 [Flush]: 商品支架:2 ↔ 商品支架:8
## Named parameters: d26_d21 = 0 mm, d27_d22 = 0 mm, d28_d21 = 0 mm, d29_d22 = 0 mm, d42_d37 = 0 mm, d43_d38 = 0 mm, d44_d37 = 0 mm, d45_d38 = 0 mm, d66_d52 = 0 mm, d67_d53 = 0 mm, d70_d56 = 0 mm, d71_d58 = 0 mm, d72_d59 = 0 mm, d75_d62 = 0 mm, d76_d52 = 0 mm, d77_d53 = 0 mm, d80_d56 = 0 mm, d81_d58 = 0 mm, d82_d59 = 0 mm, d85_d62 = 0 mm, d158_d154 = 0 mm, d159_d155 = 0 mm, d160_d154 = 0 mm, d161_d155 = 0 mm, d162_d154 = 0 mm, d163_d155 = 0 mm, d164_d154 = 0 mm, d165_d155 = 0 mm, d166_d154 = 0 mm, d167_d155 = 0 mm, d168_d154 = 0 mm, d169_d155 = 0 mm, d170_d154 = 0 mm, d171_d155 = 0 mm, d172_d154 = 0 mm, d173_d155 = 0 mm, d484_d477 = 0 mm, d485_d478 = 0 mm, d486_d479 = 0 mm, d487_d480 = 0 mm, d488_d481 = 0 mm, d489_d482 = 0 mm, d490_d483 = 0 mm, d491_d476 = 0 mm, d492_d477 = 0 mm, d493_d478 = 0 mm, d494_d479 = 0 mm, d495_d480 = 0 mm, d496_d481 = 0 mm, d497_d482 = 0 mm, d498_d483 = 0 mm, d499_d476 = 0 mm
